# Autodesk Inventor assembly: carkifelek-ass-final
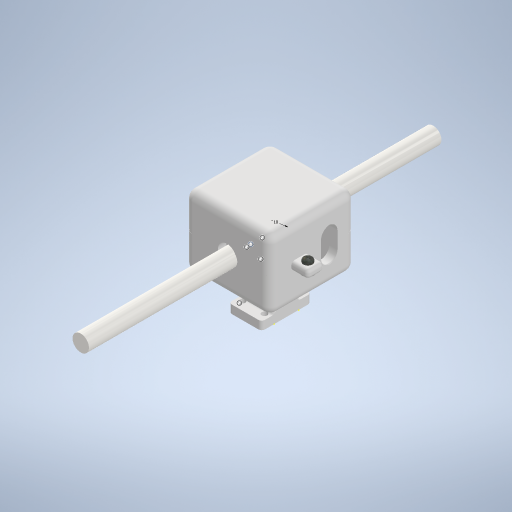
[picture p0: Inventor's stored thumbnail of the model, 512x512]
Saved by Autodesk Inventor 2023.2 (Build 272271000, 271)
## iProperties
Created: 2023-03-29
Part Number: carkifelek-ass-final
Document SubType Name: Assembly
Designer: sarp1
Author: sarp1
## Documents named in this file (9)
- C:\Users\sarp1\Documents\carkifelek-final\carkifelek-ass-final.iam
- C:\Users\sarp1\Documents\carkifelek-final\kab-f.ipt
- C:\Users\sarp1\Documents\carkifelek-final\dondurgec-b.ipt
- C:\Users\sarp1\Documents\carkifelek-final\Spur Gear11.ipt
- C:\Users\sarp1\Documents\carkifelek-final\Spur Gear21.ipt
- C:\Users\sarp1\Documents\carkifelek-final\dondurgec-a.ipt
- C:\Users\sarp1\Documents\carkifelek-final\kab-f - u_MIR1.ipt
- C:\Users\sarp1\Documents\Inventor\Content Center Files\R2023\en-US\ISO 7045  H\ISO 7045 - M3 x 6_ - 4.8 - H - ISO.ipt
- C:\Users\sarp1\Documents\Inventor\Content Center Files\R2023\en-US\ISO 7089\ISO 7089 - 3 - 140 HV(1).ipt
## Components (12 placed, 8 different names)
1. kab-f:1 — Cylindrical:1, Mate:1, Mate:2, Mate:4, Mate:5
2. dondurgec-b:1 — Rotational:1, Rotational:2, Rotational:3
3. kucuk:1 — Rotational:2
4. boyuk:1 — Rotational:1, Cylindrical:1
5. kucuk:2 — Rotational:3, Rotational:7
6. dondurgec-a:1 — Rotational:4, Rotational:5, Rotational:6, Rotational:7
7. boyuk:2 — Rotational:4
8. kucuk:3 — Rotational:5
9. kucuk:4 — Rotational:6
10. kab-f - u_MIR1:1 — Mate:1, Mate:3
11. ISO 7045 H M3 x 6 - 4.8 - H:1 — Mate:2, Mate:3
12. ISO 7089 3:1 — Mate:4, Mate:5
## Relationships (13: RevoluteJoint 7, Mate 5, CylindricalJoint 1)
- Rotational:1 [RevoluteJoint]: dondurgec-b:1 ↔ boyuk:1
- Rotational:2 [RevoluteJoint]: dondurgec-b:1 ↔ kucuk:1
- Rotational:3 [RevoluteJoint]: dondurgec-b:1 ↔ kucuk:2
- Rotational:4 [RevoluteJoint]: dondurgec-a:1 ↔ boyuk:2
- Rotational:5 [RevoluteJoint]: dondurgec-a:1 ↔ kucuk:3
- Rotational:6 [RevoluteJoint]: dondurgec-a:1 ↔ kucuk:4
- Rotational:7 [RevoluteJoint]: kucuk:2 ↔ dondurgec-a:1
- Cylindrical:1: kab-f:1 ↔ boyuk:1
- Mate:1: kab-f:1 ↔ kab-f - u_MIR1:1
- Mate:2: kab-f:1 ↔ ISO 7045 H M3 x 6 - 4.8 - H:1
- Mate:3: kab-f - u_MIR1:1 ↔ ISO 7045 H M3 x 6 - 4.8 - H:1
- Mate:4: kab-f:1 ↔ ISO 7089 3:1
- Mate:5: kab-f:1 ↔ ISO 7089 3:1
